# Autodesk Inventor assembly: 193992 DSNU-32-60-PPS-A---(60PPSA---00--0-------0)_MIR
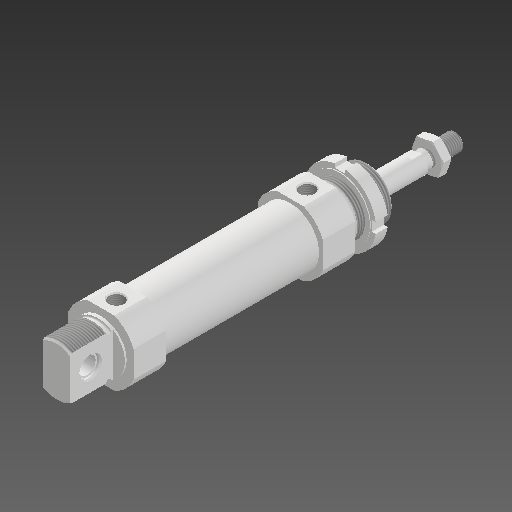
[picture p0: Inventor's stored thumbnail of the model, 512x512]
Saved by Autodesk Inventor 2021 (Build 250183000, 183)
## iProperties
Category: PARTsolutions
Company: FESTO
Part Number: 193992 DSNU-32-60-PPS-A---(60PPSA---00--0-------0)_MIR
Catalog Web Link: www.cadenas.de
Description: DSNU (m)-Round cylinder, Modular system
Vendor: FESTO
Document SubType Name: Assembly
Designer: maaro
Manufacturer: FESTO
Mass: 123.415 g
Surface Area: 454.214 cm^2
Volume: 123.415 cm^3
Density: 1 g/cm^3
Title: 193992 DSNU-32-60-PPS-A
Author: Cadenas PARTsolutions
Comments: Round cylinder, Modular system
PSOL_IDENT_0: {ATYP=ASSISTANT},{DATA=script=$CADENAS_DATA/23d-libs/festo/webfesto.vbb/&M_FAMILY=DSNU&M_GROUP=01&M_
PSOL_IDENT_1: PARTNO=193992&IDCODE1=DSNU-32-60-PPS-A&IDCODE2=&C_DSNU_DM=32&C_DSNU_HEAD=DSNU&HUB=60&M_AA=A&M_DAA=PP
PSOL_IDENT_2: S&S_SMS=N&VCSD_UPDATE_YYIDENT11=DSNU-32-60-PPS-A&customer_number_cns=&MATES=1&LOD=HI&LOCKERP=1}
NB: 193992 DSNU-32-60-PPS-A---(60PPSA---00--0-------0)
NN: DSNU (m)
NT: Round cylinder, Modular system
NBSYN: $TNR. $IDCODE1.---($HUB.$DA.$PE.$ZD.$VS.$KA.$K2A.$K6.$K3.$K5.$K8.$KP.$R3.$R8.$TB.$KS.$LS.$ATEX.$HUBST.)
LINA: 193992 DSNU-32-60-PPS-A
CATALOG: Festo
OFFICIAL_STANDARD_NUMBERS: ISO 6432
TNR: 193992
TYP: DSNU-32
KDM: 32
HUB: 60
HUBST: 0
DA: PPS
PE: A
ZD: -
VS: -
KA: -
K2A: 0
K6: 0
K3: -
K5: -
K8: 0
KP: -
R3: -
R8: -
TB: -
KS: -
LS: -
ATEX: -
A1: 35
A2: 500
A3: 8
A4: 55.5
AB: 30
AM: 22
B: 30
BB: 4
BE: M30x1,5
BS: 6.6
B1: 48
B2: 10
B3: 30
B4: 9
B5: 25
B6: 11
B7: 3
CD: 10
D: 38
D1: 30
D2: 12
D3: 33.6
D4: 10
D5: 34
D6: 42
D7: 30
EE: G1/8
EW: 16
F: 38
FF: M5
F1: 19
H: 40
H1: 6
KK: M10x1.25
K1: M6
K2: 2.5
KV: 0
KW: 8
KV2: 17
KW2: 5
L: 13
LH: 12
LK: 15
L1: 189.5
L2: 129.5
L3: 9
L4: 26
L5: 24
L6: 56
L7: 30
L8: 19
L9: 25
L10: 85.5
L11: 97.5
L12: 65.5
L13: 137.5
ST: 6.8
SW: 10
T: 12
WH: 34
X: 2.6
XC: 177.5
SUPPLIER: FESTO
ARTICLENO: 193992 DSNU-32-60-PPS-A---(60PPSA---00--0-------0)
BOMINFO: 193992 DSNU-32-60-PPS-A
CREATOR: CADENAS GmbH
## Documents named in this file (5)
- C:\Users\maaro\Documents\UNAL\Automatización de Procesos de Manufactura\Github\Proyecto_APM\CADs estaciones a automatizar\Estación corte\193992 DSNU-32-60-PPS-A---(60PPSA---00--0-------0)_MIR.iam
- C:\Users\maaro\Documents\UNAL\Automatización de Procesos de Manufactura\Github\Proyecto_APM\CADs estaciones a automatizar\Estación corte\193992 DSNU-32-60-PPS---(A----0-ZR)_MIR.ipt
- C:\Users\maaro\Documents\UNAL\Automatización de Procesos de Manufactura\Github\Proyecto_APM\CADs estaciones a automatizar\Estación corte\3753 M30x1_5_MIR.ipt
- C:\Users\maaro\Documents\UNAL\Automatización de Procesos de Manufactura\Github\Proyecto_APM\CADs estaciones a automatizar\Estación corte\193992 DSNU-32-60-PPS---(A---00--0-KS)_MIR.ipt
- C:\Users\maaro\Documents\UNAL\Automatización de Procesos de Manufactura\Github\Proyecto_APM\CADs estaciones a automatizar\Estación corte\DIN-439-B - M10x1_25(F)_MIR.ipt
## Components (4 placed, 4 different names)
1. 193992 DSNU-32-60-PPS---(A----0-ZR)_MIR:1 — Mate:3, Cylindrical:1
2. 3753 M30x1_5_MIR:1
3. 193992 DSNU-32-60-PPS---(A---00--0-KS)_MIR:1 — Mate:3, NUT1_XY@3 <-> 2CYL_XY@4, NUT1_Z@3 <-> 2CYL_Z@4, NUT1_YZ@3 <-> 2CYL_YZ@4, Cylindrical:1
4. DIN-439-B - M10x1_25(F)_MIR:1 — NUT1_XY@3 <-> 2CYL_XY@4, NUT1_Z@3 <-> 2CYL_Z@4, NUT1_YZ@3 <-> 2CYL_YZ@4
## Relationships (5: Mate 3, Angle 1, CylindricalJoint 1)
- Mate:3: 193992 DSNU-32-60-PPS---(A----0-ZR)_MIR:1 ↔ 193992 DSNU-32-60-PPS---(A---00--0-KS)_MIR:1
- NUT1_XY@3 <-> 2CYL_XY@4 [Mate] (6.267 mm): 193992 DSNU-32-60-PPS---(A---00--0-KS)_MIR:1 ↔ DIN-439-B - M10x1_25(F)_MIR:1
- NUT1_Z@3 <-> 2CYL_Z@4 [Mate]: 193992 DSNU-32-60-PPS---(A---00--0-KS)_MIR:1 ↔ DIN-439-B - M10x1_25(F)_MIR:1
- NUT1_YZ@3 <-> 2CYL_YZ@4 [Angle] (0 deg): 193992 DSNU-32-60-PPS---(A---00--0-KS)_MIR:1 ↔ DIN-439-B - M10x1_25(F)_MIR:1
- Cylindrical:1: 193992 DSNU-32-60-PPS---(A----0-ZR)_MIR:1 ↔ 193992 DSNU-32-60-PPS---(A---00--0-KS)_MIR:1
